# Autodesk Inventor assembly: R-W v6
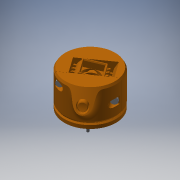
[picture p0: Inventor's stored thumbnail of the model, 180x180]
Saved by Autodesk Inventor 2018.2 (Build 222227000, 227)
## iProperties
Created: 2017-09-22
Part Number: R-W v6
Material: 一般
Document SubType Name: Assembly
Designer: sktom
Author: sktom
## Documents named in this file (14)
- D:\CloudStrage\OneDrive\CADMech\HbSizeMMech\UnitWrist\Unit_MR-W.iam
- D:\CloudStrage\OneDrive\CADMech\HbSizeMMech\UnitWrist\MR-W-02.ipt
- D:\CloudStrage\OneDrive\CADMech\HbSizeMMech\UnitWrist\MR-W-01.ipt
- D:\CloudStrage\OneDrive\CADMech\HbSizeMMech\UnitWrist\MR-W-04.ipt
- D:\CloudStrage\OneDrive\CADMech\HbSizeMMech\UnitWrist\MR-W-05.ipt
- D:\CloudStrage\OneDrive\CADMech\HbSizeMMech\UnitWrist\MR-W-06.ipt
- D:\CloudStrage\OneDrive\CADMech\HbSizeMMech\UnitWrist\MR-W-07.ipt
- D:\CloudStrage\OneDrive\CADMech\HbSizeMMech\UnitWrist\MR-W-08.ipt
- D:\CloudStrage\OneDrive\CADMech\HbSizeMMech\UnitWrist\MR-W-03.ipt
- D:\CloudStrage\OneDrive\CADMech\HbSizeMMech\UnitWrist\Parts_FlatScrew_M2_L6.ipt
- D:\CloudStrage\OneDrive\CADMech\HbSizeMMech\UnitWrist\Parts_Screw_M3_L6.ipt
- D:\CloudStrage\OneDrive\CADMech\HbSizeMMech\UnitWrist\Parts_Screw_M2_L8.ipt
- D:\CloudStrage\OneDrive\CADMech\HbSizeMMech\UnitWrist\Parts_BallBearing_SBM-SUJ-5.5.ipt
- D:\CloudStrage\OneDrive\CADMech\HbSizeMMech\UnitWrist\Parts_CoilSpring_CP 0.6-5.5-8.ipt
## Components (21 placed, 13 different names)
1. MR-W-01:1 — 挿入:12, メイト:1
2. MR-W-02:1 — 挿入:8, 円柱状:1, 円柱状:2, フラッシュ:1, 挿入:12, メイト:1, 挿入:14, メイト:2, 挿入:15, 挿入:16, 挿入:20, 挿入:21, 挿入:22
3. MR-W-03:1 — 円柱状:1, 円柱状:2, フラッシュ:1
4. MR-W-04:1 — 挿入:1, 挿入:2, 挿入:5, 挿入:6, 挿入:7, 挿入:8
5. MR-W-05:1 — 挿入:1, 挿入:2, 挿入:3, 挿入:4
6. MR-W-06:1 — 挿入:14, 円柱状:3, 挿入:19
7. MR-W-07:1 — 円柱状:3, メイト:2
8. MR-W-08:1 — 挿入:15, 挿入:16, 挿入:17, 挿入:18
9. Parts_BallBearing_SBM-SUJ-5.5:1
10. Parts_BallBearing_SBM-SUJ-5.5:2
11. Parts_CoilSpring_CP 0.6-5.5-8:2 — 挿入:20
12. Parts_CoilSpring_CP 0.6-5.5-8:3 — 挿入:22
13. Parts_CoilSpring_CP 0.6-5.5-8:4 — 挿入:21
14. Parts_CoilSpring_CP 0.6-5.5-8:1 — 挿入:19
15. Parts_FlatScrew_M2_L6:1 — 挿入:4
16. Parts_FlatScrew_M2_L6:2 — 挿入:3
17. Parts_Screw_M2_L8:1 — 挿入:6
18. Parts_Screw_M2_L8:2 — 挿入:7
19. Parts_Screw_M2_L8:3 — 挿入:5
20. Parts_Screw_M3_L6:1 — 挿入:18
21. Parts_Screw_M3_L6:2 — 挿入:17
## Relationships (24: Insert 18, CylindricalJoint 3, Mate 2, Flush 1)
- 挿入:1 [Insert]: MR-W-04:1 ↔ MR-W-05:1
- 挿入:2 [Insert]: MR-W-04:1 ↔ MR-W-05:1
- 挿入:3 [Insert]: MR-W-05:1 ↔ Parts_FlatScrew_M2_L6:2
- 挿入:4 [Insert]: MR-W-05:1 ↔ Parts_FlatScrew_M2_L6:1
- 挿入:5 [Insert]: MR-W-04:1 ↔ Parts_Screw_M2_L8:3
- 挿入:6 [Insert]: MR-W-04:1 ↔ Parts_Screw_M2_L8:1
- 挿入:7 [Insert]: MR-W-04:1 ↔ Parts_Screw_M2_L8:2
- 挿入:8 [Insert]: MR-W-02:1 ↔ MR-W-04:1
- 円柱状:1 [CylindricalJoint]: MR-W-02:1 ↔ MR-W-03:1
- 円柱状:2 [CylindricalJoint]: MR-W-02:1 ↔ MR-W-03:1
- フラッシュ:1 [Flush]: MR-W-02:1 ↔ MR-W-03:1
- 挿入:12 [Insert]: MR-W-01:1 ↔ MR-W-02:1
- メイト:1 [Mate] (0.265 mm): MR-W-01:1 ↔ MR-W-02:1
- 挿入:14 [Insert]: MR-W-02:1 ↔ MR-W-06:1
- 円柱状:3 [CylindricalJoint]: MR-W-06:1 ↔ MR-W-07:1
- メイト:2 [Mate]: MR-W-02:1 ↔ MR-W-07:1
- 挿入:15 [Insert]: MR-W-02:1 ↔ MR-W-08:1
- 挿入:16 [Insert]: MR-W-02:1 ↔ MR-W-08:1
- 挿入:17 [Insert]: MR-W-08:1 ↔ Parts_Screw_M3_L6:2
- 挿入:18 [Insert]: MR-W-08:1 ↔ Parts_Screw_M3_L6:1
- 挿入:19 [Insert]: MR-W-06:1 ↔ Parts_CoilSpring_CP 0.6-5.5-8:1
- 挿入:20 [Insert]: MR-W-02:1 ↔ Parts_CoilSpring_CP 0.6-5.5-8:2
- 挿入:21 [Insert]: MR-W-02:1 ↔ Parts_CoilSpring_CP 0.6-5.5-8:4
- 挿入:22 [Insert]: MR-W-02:1 ↔ Parts_CoilSpring_CP 0.6-5.5-8:3
